# Autodesk Inventor assembly: RaspberryPi
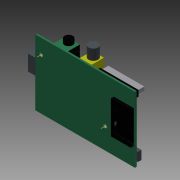
[picture p0: Inventor's stored thumbnail of the model, 180x180]
Saved by Autodesk Inventor 2014 (Build 180170000, 170)
## iProperties
Created: 2013-05-24
Part Number: RaspberryPi
Document SubType Name: Assembly
Designer: hartmann
Author: hartmann
## Documents named in this file (2)
- C:\Users\Felix\Desktop\Beep\Hardware\3D-CAD\parts\electronic\RaspberryPi\RaspberryPi.iam
- C:\Users\Felix\Desktop\Beep\Hardware\3D-CAD\parts\electronic\RaspberryPi\PCB.ipt
## Components (1 placed, 1 different names)
1. PCB:1 — Passend:1, Passend:2
## Relationships (2: Mate 2)
- Passend:1 [Mate]: PCB:1
- Passend:2 [Mate]: PCB:1
